# Autodesk Inventor assembly: Board_Final
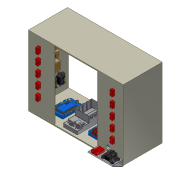
[picture p0: Inventor's stored thumbnail of the model, 180x180]
Saved by Autodesk Inventor 2012 (Build 160160000, 160)
## iProperties
Created: 2012-02-05
Part Number: Board_Final
Document SubType Name: Assembly
Designer: JesseK
Mass: 6783.94 g
Surface Area: 21973 cm^2
Volume: 6496.43 cm^3
Density: 1.04426 g/cm^3
Author: JesseK
## Documents named in this file (10)
- Z:\UserData\Documents\Inventor\team1885frc\Robot2012\Electronics Board\Board_Final.iam
- Z:\UserData\Documents\Inventor\team1885frc\Robot2012\Electronics Board\Board_Final_Concept.ipt
- Z:\UserData\Documents\Inventor\team1885frc\Electronics\cRIO_4Slot\Imported Components\cu_crio-9075_4-slot\cu_crio-9075_4-slot.ipt
- Z:\UserData\Documents\Inventor\team1885frc\Electronics\DigitalSidecar\elc_Digital_Sidecar_inv.iam
- Z:\UserData\Documents\Inventor\team1885frc\Electronics\Jag\Jag.iam
- Z:\UserData\Documents\Inventor\team1885frc\Electronics\spike relay\Spike_Assem.iam
- Z:\UserData\Documents\Inventor\team1885frc\Electronics\PowerDistributionBoard\elc_Power_Distro_inv.iam
- Z:\UserData\Documents\Inventor\team1885frc\Electronics\elc_Battery_Plug_inv.ipt
- Z:\UserData\Documents\Inventor\team1885frc\Robot2012\Electronics Board\BatteryMount.ipt
- Z:\UserData\Documents\Inventor\team1885frc\Electronics\Breaker\Breaker.iam
## Components (29 placed, 9 different names)
1. Board_Final_Concept:1 — Mate:1, Mate:2, Mate:4, Mate:5, Mate:6, Mate:7, Mate:8, Mate:9, Mate:10, Mate:11, Mate:12, Mate:13, Mate:14, Mate:15, Mate:16, Mate:17, Mate:18, Flush:1, Flush:5, Mate:22, Mate:23, Mate:24, Mate:25, Mate:26, Mate:27, Mate:28, Mate:30, Mate:31, Mate:32, Mate:33, Mate:34, Mate:35, Mate:36, Mate:37, Mate:38, Mate:43, Mate:44, Mate:45, Mate:46, Mate:51, Mate:52, Mate:53, Flush:7
2. cu_crio-9075_4-slot:1 — Mate:13
3. elc_Digital_Sidecar_inv:1 [sub-assembly] — Mate:11, Mate:14
4. Jag:1 [sub-assembly] — Mate:12, Flush:5
5. Jag:2 [sub-assembly] — Mate:4
6. Jag:3 [sub-assembly] — Mate:5
7. Jag:4 [sub-assembly] — Mate:9
8. Jag:5 [sub-assembly] — Mate:6
9. Jag:6 [sub-assembly] — Mate:7
10. Jag:7 [sub-assembly] — Mate:8
11. Jag:8 [sub-assembly] — Mate:10
12. Spike_Assem:1 [sub-assembly] — Mate:15, Mate:21, Flush:2, Flush:3
13. Spike_Assem:2 [sub-assembly] — Mate:16, Mate:19, Mate:20, Flush:4
14. Spike_Assem:3 [sub-assembly] — Mate:17, Mate:20, Flush:3, Flush:4
15. Spike_Assem:4 [sub-assembly] — Mate:18, Mate:19, Flush:1, Mate:21, Flush:2
16. elc_Power_Distro_inv:1 [sub-assembly] — Mate:1, Mate:2
17. elc_Battery_Plug_inv:1 — Mate:22, Mate:23, Mate:50
18. elc_Battery_Plug_inv:2 — Mate:24, Mate:43, Mate:49, Mate:50
19. elc_Battery_Plug_inv:3 — Mate:25, Mate:44, Mate:48, Mate:49
20. elc_Battery_Plug_inv:4 — Mate:26, Mate:45, Mate:47, Mate:48
21. elc_Battery_Plug_inv:5 — Mate:27, Mate:46, Mate:47
22. elc_Battery_Plug_inv:6 — Mate:33, Mate:35, Mate:41, Mate:42
23. elc_Battery_Plug_inv:7 — Mate:31, Mate:37, Mate:39, Mate:40
24. elc_Battery_Plug_inv:8 — Mate:32, Mate:38, Mate:39
25. elc_Battery_Plug_inv:11 — Mate:28, Mate:34, Mate:42
26. elc_Battery_Plug_inv:12 — Mate:30, Mate:36, Mate:40, Mate:41
27. BatteryMount:1 — Mate:51, Mate:52, Mate:53, Mate:54, Flush:6, Mate:55
28. Breaker:1 [sub-assembly] — Mate:54, Flush:6
29. elc_Battery_Plug_inv:13 — Mate:55, Flush:7
## Relationships (60: Mate 53, Flush 7)
- Mate:1 (50.8 mm): Board_Final_Concept:1 ↔ elc_Power_Distro_inv:1
- Mate:2: Board_Final_Concept:1 ↔ elc_Power_Distro_inv:1
- Mate:4: Board_Final_Concept:1 ↔ Jag:2
- Mate:5: Board_Final_Concept:1 ↔ Jag:3
- Mate:6: Board_Final_Concept:1 ↔ Jag:5
- Mate:7: Board_Final_Concept:1 ↔ Jag:6
- Mate:8: Board_Final_Concept:1 ↔ Jag:7
- Mate:9: Board_Final_Concept:1 ↔ Jag:4
- Mate:10: Board_Final_Concept:1 ↔ Jag:8
- Mate:11: Board_Final_Concept:1 ↔ elc_Digital_Sidecar_inv:1
- Mate:12: Board_Final_Concept:1 ↔ Jag:1
- Mate:13: Board_Final_Concept:1 ↔ cu_crio-9075_4-slot:1
- Mate:14 (76.2 mm): Board_Final_Concept:1 ↔ elc_Digital_Sidecar_inv:1
- Mate:15: Board_Final_Concept:1 ↔ Spike_Assem:1
- Mate:16: Board_Final_Concept:1 ↔ Spike_Assem:2
- Mate:17: Board_Final_Concept:1 ↔ Spike_Assem:3
- Mate:18: Board_Final_Concept:1 ↔ Spike_Assem:4
- Mate:19: Spike_Assem:2 ↔ Spike_Assem:4
- Flush:1 (50.8 mm): Board_Final_Concept:1 ↔ Spike_Assem:4
- Mate:20: Spike_Assem:2 ↔ Spike_Assem:3
- Mate:21: Spike_Assem:1 ↔ Spike_Assem:4
- Flush:2 (50.8 mm): Spike_Assem:1 ↔ Spike_Assem:4
- Flush:3 (-50.8 mm): Spike_Assem:1 ↔ Spike_Assem:3
- Flush:4 (-50.8 mm): Spike_Assem:2 ↔ Spike_Assem:3
- Flush:5 (76.2 mm): Board_Final_Concept:1 ↔ Jag:1
- Mate:22: Board_Final_Concept:1 ↔ elc_Battery_Plug_inv:1
- Mate:23: Board_Final_Concept:1 ↔ elc_Battery_Plug_inv:1
- Mate:24: Board_Final_Concept:1 ↔ elc_Battery_Plug_inv:2
- Mate:25: Board_Final_Concept:1 ↔ elc_Battery_Plug_inv:3
- Mate:26: Board_Final_Concept:1 ↔ elc_Battery_Plug_inv:4
- Mate:27: Board_Final_Concept:1 ↔ elc_Battery_Plug_inv:5
- Mate:28: Board_Final_Concept:1 ↔ elc_Battery_Plug_inv:11
- Mate:30: Board_Final_Concept:1 ↔ elc_Battery_Plug_inv:12
- Mate:31: Board_Final_Concept:1 ↔ elc_Battery_Plug_inv:7
- Mate:32: Board_Final_Concept:1 ↔ elc_Battery_Plug_inv:8
- Mate:33: Board_Final_Concept:1 ↔ elc_Battery_Plug_inv:6
- Mate:34: Board_Final_Concept:1 ↔ elc_Battery_Plug_inv:11
- Mate:35: Board_Final_Concept:1 ↔ elc_Battery_Plug_inv:6
- Mate:36: Board_Final_Concept:1 ↔ elc_Battery_Plug_inv:12
- Mate:37: Board_Final_Concept:1 ↔ elc_Battery_Plug_inv:7
- Mate:38: Board_Final_Concept:1 ↔ elc_Battery_Plug_inv:8
- Mate:39: elc_Battery_Plug_inv:7 ↔ elc_Battery_Plug_inv:8
- Mate:40: elc_Battery_Plug_inv:7 ↔ elc_Battery_Plug_inv:12
- Mate:41: elc_Battery_Plug_inv:6 ↔ elc_Battery_Plug_inv:12
- Mate:42: elc_Battery_Plug_inv:6 ↔ elc_Battery_Plug_inv:11
- Mate:43: Board_Final_Concept:1 ↔ elc_Battery_Plug_inv:2
- Mate:44: Board_Final_Concept:1 ↔ elc_Battery_Plug_inv:3
- Mate:45: Board_Final_Concept:1 ↔ elc_Battery_Plug_inv:4
- Mate:46: Board_Final_Concept:1 ↔ elc_Battery_Plug_inv:5
- Mate:47: elc_Battery_Plug_inv:4 ↔ elc_Battery_Plug_inv:5
- Mate:48: elc_Battery_Plug_inv:3 ↔ elc_Battery_Plug_inv:4
- Mate:49: elc_Battery_Plug_inv:2 ↔ elc_Battery_Plug_inv:3
- Mate:50: elc_Battery_Plug_inv:1 ↔ elc_Battery_Plug_inv:2
- Mate:51: Board_Final_Concept:1 ↔ BatteryMount:1
- Mate:52 (-31.75 mm): Board_Final_Concept:1 ↔ BatteryMount:1
- Mate:53: Board_Final_Concept:1 ↔ BatteryMount:1
- Mate:54: BatteryMount:1 ↔ Breaker:1
- Flush:6 (6.35 mm): BatteryMount:1 ↔ Breaker:1
- Mate:55: BatteryMount:1 ↔ elc_Battery_Plug_inv:13
- Flush:7 (-63.5 mm): Board_Final_Concept:1 ↔ elc_Battery_Plug_inv:13
